# Autodesk Inventor assembly: mesa_suporte_de_placa_automatica
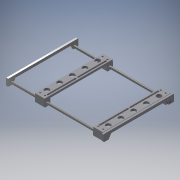
[picture p0: Inventor's stored thumbnail of the model, 180x180]
Saved by Autodesk Inventor 2018 (Build 220112000, 112)
## iProperties
Created: 2018-05-17
Part Number: mesa_suporte_de_placa_automatica
Material: Genérico
Document SubType Name: Assembly
Designer: Usuario
Mass: 2681.39 g
Surface Area: 5192.59 cm^2
Volume: 1283.96 cm^3
Density: 2.08838 g/cm^3
Author: Usuario
## Documents named in this file (8)
- C:\Users\Georgines\Documents\EstacaoBGA\Peças 3D\mesa_suporte_de_placa_automatica.iam
- C:\Users\Georgines\Documents\EstacaoBGA\Peças 3D\guia_linear_12mm.ipt
- C:\Users\Georgines\Documents\EstacaoBGA\Peças 3D\SBR12UU.iam
- C:\Users\Georgines\Documents\EstacaoBGA\Peças 3D\EsbarrosCarro.ipt
- C:\Users\Georgines\Documents\EstacaoBGA\Peças 3D\SuportePincas.ipt
- C:\Users\Georgines\Documents\EstacaoBGA\Peças 3D\Peça1.ipt
- C:\Users\Georgines\Documents\EstacaoBGA\Peças 3D\blocoRolamentoLinearCarroMesa.iam
- C:\Users\Georgines\Documents\EstacaoBGA\Peças 3D\SuportePincasBlocoFabricado.ipt
## Components (17 placed, 7 different names)
1. guia_linear_12mm:1 — Coincidência:4, Coincidência:27, Coincidência:28, Coincidência:31, Coincidência:40, Alinhamento:28, Coincidência:41, Coincidência:43, Alinhamento:39, Alinhamento:40
2. guia_linear_12mm:2 — Coincidência:4, Coincidência:29, Coincidência:30, Coincidência:32, Alinhamento:23, Coincidência:39, Coincidência:42, Coincidência:44, Alinhamento:38, Alinhamento:41
3. SBR12UU:1 [sub-assembly] — Coincidência:28, Alinhamento:18, Alinhamento:19, Coincidência:38, Alinhamento:26, Alinhamento:27
4. SBR12UU:2 [sub-assembly] — Coincidência:29, Alinhamento:18, Alinhamento:19
5. SBR12UU:3 [sub-assembly] — Coincidência:27, Alinhamento:20, Alinhamento:21, Coincidência:37, Alinhamento:24, Alinhamento:25
6. SBR12UU:4 [sub-assembly] — Coincidência:30, Alinhamento:20, Alinhamento:21
7. EsbarrosCarro:2 — Coincidência:31, Coincidência:32, Alinhamento:23, Alinhamento:40, Alinhamento:41, Coincidência:47
8. SuportePincas:2 — Coincidência:38, Alinhamento:26, Alinhamento:27
9. SuportePincas:3 — Coincidência:37, Alinhamento:24, Alinhamento:25, Alinhamento:29
10. EsbarrosCarro:3 — Coincidência:39, Coincidência:40, Alinhamento:28, Alinhamento:38, Alinhamento:39, Coincidência:48
11. PCB — Alinhamento:29
12. blocoRolamentoLinearCarroMesa:1 [sub-assembly] — Coincidência:41, Alinhamento:30, Alinhamento:31, Coincidência:46, Alinhamento:36, Alinhamento:37, Coincidência:47
13. blocoRolamentoLinearCarroMesa:2 [sub-assembly] — Coincidência:42, Alinhamento:30, Alinhamento:31
14. blocoRolamentoLinearCarroMesa:3 [sub-assembly] — Coincidência:44, Alinhamento:32, Alinhamento:33
15. blocoRolamentoLinearCarroMesa:4 [sub-assembly] — Coincidência:43, Alinhamento:32, Alinhamento:33, Coincidência:45, Alinhamento:34, Alinhamento:35, Coincidência:48
16. SuportePincasBlocoFabricado:1 — Coincidência:46, Alinhamento:36, Alinhamento:37
17. SuportePincasBlocoFabricado:3 — Coincidência:45, Alinhamento:34, Alinhamento:35
## Relationships (42: Flush 23, Mate 19)
- Coincidência:4 [Mate]: guia_linear_12mm:1 ↔ guia_linear_12mm:2
- Coincidência:27 [Mate]: guia_linear_12mm:1 ↔ SBR12UU:3
- Coincidência:28 [Mate]: guia_linear_12mm:1 ↔ SBR12UU:1
- Coincidência:29 [Mate]: guia_linear_12mm:2 ↔ SBR12UU:2
- Coincidência:30 [Mate]: guia_linear_12mm:2 ↔ SBR12UU:4
- Alinhamento:18 [Flush]: SBR12UU:1 ↔ SBR12UU:2
- Alinhamento:19 [Flush]: SBR12UU:1 ↔ SBR12UU:2
- Alinhamento:20 [Flush]: SBR12UU:3 ↔ SBR12UU:4
- Alinhamento:21 [Flush]: SBR12UU:3 ↔ SBR12UU:4
- Coincidência:31 [Mate]: guia_linear_12mm:1 ↔ EsbarrosCarro:2
- Coincidência:32 [Mate]: guia_linear_12mm:2 ↔ EsbarrosCarro:2
- Alinhamento:23 [Flush]: guia_linear_12mm:2 ↔ EsbarrosCarro:2
- Coincidência:37 [Mate]: SBR12UU:3 ↔ SuportePincas:3
- Alinhamento:24 [Flush]: SBR12UU:3 ↔ SuportePincas:3
- Alinhamento:25 [Flush]: SBR12UU:3 ↔ SuportePincas:3
- Coincidência:38 [Mate]: SBR12UU:1 ↔ SuportePincas:2
- Alinhamento:26 [Flush]: SBR12UU:1 ↔ SuportePincas:2
- Alinhamento:27 [Flush]: SBR12UU:1 ↔ SuportePincas:2
- Coincidência:39 [Mate]: guia_linear_12mm:2 ↔ EsbarrosCarro:3
- Coincidência:40 [Mate]: guia_linear_12mm:1 ↔ EsbarrosCarro:3
- Alinhamento:28 [Flush]: guia_linear_12mm:1 ↔ EsbarrosCarro:3
- Alinhamento:29 [Flush]: SuportePincas:3 ↔ PCB
- Coincidência:41 [Mate]: guia_linear_12mm:1 ↔ blocoRolamentoLinearCarroMesa:1
- Coincidência:42 [Mate]: guia_linear_12mm:2 ↔ blocoRolamentoLinearCarroMesa:2
- Coincidência:43 [Mate]: guia_linear_12mm:1 ↔ blocoRolamentoLinearCarroMesa:4
- Coincidência:44 [Mate]: guia_linear_12mm:2 ↔ blocoRolamentoLinearCarroMesa:3
- Alinhamento:30 [Flush]: blocoRolamentoLinearCarroMesa:1 ↔ blocoRolamentoLinearCarroMesa:2
- Alinhamento:31 [Flush]: blocoRolamentoLinearCarroMesa:1 ↔ blocoRolamentoLinearCarroMesa:2
- Alinhamento:32 [Flush]: blocoRolamentoLinearCarroMesa:3 ↔ blocoRolamentoLinearCarroMesa:4
- Alinhamento:33 [Flush]: blocoRolamentoLinearCarroMesa:3 ↔ blocoRolamentoLinearCarroMesa:4
- Coincidência:45 [Mate]: blocoRolamentoLinearCarroMesa:4 ↔ SuportePincasBlocoFabricado:3
- Alinhamento:34 [Flush]: blocoRolamentoLinearCarroMesa:4 ↔ SuportePincasBlocoFabricado:3
- Alinhamento:35 [Flush]: blocoRolamentoLinearCarroMesa:4 ↔ SuportePincasBlocoFabricado:3
- Coincidência:46 [Mate]: blocoRolamentoLinearCarroMesa:1 ↔ SuportePincasBlocoFabricado:1
- Alinhamento:36 [Flush]: blocoRolamentoLinearCarroMesa:1 ↔ SuportePincasBlocoFabricado:1
- Alinhamento:37 [Flush]: blocoRolamentoLinearCarroMesa:1 ↔ SuportePincasBlocoFabricado:1
- Alinhamento:38 [Flush]: guia_linear_12mm:2 ↔ EsbarrosCarro:3
- Alinhamento:39 [Flush]: guia_linear_12mm:1 ↔ EsbarrosCarro:3
- Alinhamento:40 [Flush]: guia_linear_12mm:1 ↔ EsbarrosCarro:2
- Alinhamento:41 [Flush]: guia_linear_12mm:2 ↔ EsbarrosCarro:2
- Coincidência:47 [Mate]: EsbarrosCarro:2 ↔ blocoRolamentoLinearCarroMesa:1
- Coincidência:48 [Mate]: EsbarrosCarro:3 ↔ blocoRolamentoLinearCarroMesa:4
